# Autodesk Inventor assembly: Ensamblaje_soportme molde_barras
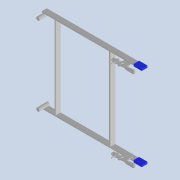
[picture p0: Inventor's stored thumbnail of the model, 180x180]
Saved by Autodesk Inventor 2021 (Build 250183000, 183)
## iProperties
Created: 2021-04-17
Part Number: Ensamblaje_soportme molde_barras
Document SubType Name: Assembly
Designer: Admin
Author: Admin
## Documents named in this file (5)
- C:\Users\Admin\OneDrive - Universidad Nacional de Colombia\Doceabo semestre\PAI\Modelados 3D\Ensamblaje_soportme molde_barras.iam
- C:\Users\Admin\OneDrive - Universidad Nacional de Colombia\Doceabo semestre\PAI\Modelados 3D\Soporte_molde.ipt
- C:\Users\Admin\OneDrive - Universidad Nacional de Colombia\Doceabo semestre\PAI\Modelados 3D\Mangas_soporte_molde.ipt
- C:\Users\Admin\OneDrive - Universidad Nacional de Colombia\Doceabo semestre\PAI\Modelados 3D\Toggle_clamp.iam
- C:\Users\Admin\OneDrive - Universidad Nacional de Colombia\Doceabo semestre\PAI\Modelados 3D\Barra_circular_soporte.ipt
## Components (7 placed, 4 different names)
1. Soporte_molde:1 — Coincidencia:1, Coincidencia:2, Coincidencia:3, Coincidencia:4, Coincidencia:5, Coincidencia:6, Coincidencia:7, Coincidencia:8, De rotación:1, De rotación:2
2. Mangas_soporte_molde:1 — Coincidencia:1, Coincidencia:2, Coincidencia:3
3. Mangas_soporte_molde:2 — Coincidencia:4, Coincidencia:5, Coincidencia:6
4. Toggle_clamp:1 [sub-assembly] — Coincidencia:7
5. Toggle_clamp:2 [sub-assembly] — Coincidencia:8
6. Barra_circular_soporte:1 — De rotación:1
7. Barra_circular_soporte:2 — De rotación:2
## Relationships (10: Mate 8, RevoluteJoint 2)
- Coincidencia:1 [Mate]: Soporte_molde:1 ↔ Mangas_soporte_molde:1
- Coincidencia:2 [Mate]: Soporte_molde:1 ↔ Mangas_soporte_molde:1
- Coincidencia:3 [Mate]: Soporte_molde:1 ↔ Mangas_soporte_molde:1
- Coincidencia:4 [Mate]: Soporte_molde:1 ↔ Mangas_soporte_molde:2
- Coincidencia:5 [Mate]: Soporte_molde:1 ↔ Mangas_soporte_molde:2
- Coincidencia:6 [Mate]: Soporte_molde:1 ↔ Mangas_soporte_molde:2
- Coincidencia:7 [Mate]: Soporte_molde:1 ↔ Toggle_clamp:1
- Coincidencia:8 [Mate]: Soporte_molde:1 ↔ Toggle_clamp:2
- De rotación:1 [RevoluteJoint]: Soporte_molde:1 ↔ Barra_circular_soporte:1
- De rotación:2 [RevoluteJoint]: Soporte_molde:1 ↔ Barra_circular_soporte:2
